# Autodesk Inventor assembly: dinolite_holder
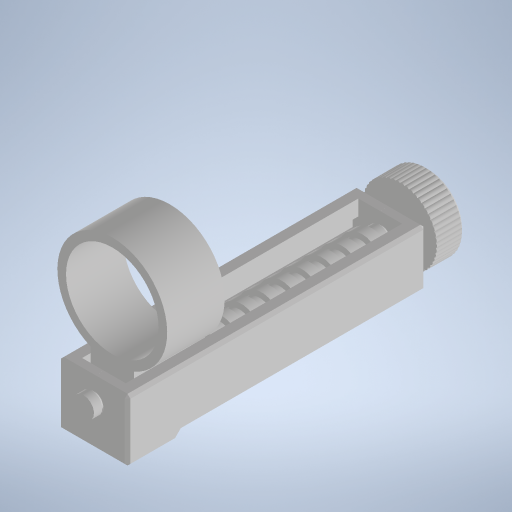
[picture p0: Inventor's stored thumbnail of the model, 512x512]
Saved by Autodesk Inventor 2024 (Build 280153000, 153)
## iProperties
Created: 2021-03-03
Part Number: dinolite_holder
Document SubType Name: Assembly
Designer: dsdan
Author: dsdan
## Documents named in this file (5)
- E:\OneDrive - Imperial College London\DragonVision_DanielKo\Instrumentation\Ephys_rig_2021\dinolite_holder.iam
- E:\OneDrive - Imperial College London\DragonVision_DanielKo\Instrumentation\Ephys_rig_2021\lead_screw_nut.ipt
- E:\OneDrive - Imperial College London\DragonVision_DanielKo\Instrumentation\Ephys_rig_2021\lead_screw_housing.ipt
- E:\OneDrive - Imperial College London\DragonVision_DanielKo\Instrumentation\Ephys_rig_2021\lead_screw.ipt
- E:\OneDrive - Imperial College London\DragonVision_DanielKo\Instrumentation\Ephys_rig_2021\lead_screw_housing_l.ipt
## Components (4 placed, 4 different names)
1. lead_screw_nut:1 — Mate:1, Angle:1, Rotation/Translation:1, Mate:4
2. lead_screw_housing:1 — Mate:2, Mate:3, Angle:1, Mate:5, Flush:1, Flush:2
3. lead_screw:1 — Mate:1, Mate:2, Mate:3, Rotation/Translation:1, Mate:4
4. lead_screw_housing_l:1 — Mate:5, Flush:1, Flush:2
## Relationships (9: Mate 5, Flush 2, Angle 1, RelateRotateTranslate 1)
- Mate:1: lead_screw_nut:1 ↔ lead_screw:1
- Mate:2: lead_screw_housing:1 ↔ lead_screw:1
- Mate:3: lead_screw_housing:1 ↔ lead_screw:1
- Angle:1 (0 deg): lead_screw_nut:1 ↔ lead_screw_housing:1
- Rotation/Translation:1 [RelateRotateTranslate] (1.5 mm): lead_screw_nut:1 ↔ lead_screw:1
- Mate:4: lead_screw_nut:1 ↔ lead_screw:1
- Mate:5: lead_screw_housing:1 ↔ lead_screw_housing_l:1
- Flush:1: lead_screw_housing:1 ↔ lead_screw_housing_l:1
- Flush:2: lead_screw_housing:1 ↔ lead_screw_housing_l:1
